# Autodesk Inventor assembly: dog_2
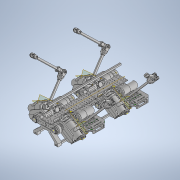
[picture p0: Inventor's stored thumbnail of the model, 180x180]
Saved by Autodesk Inventor 2020 (Build 240168000, 168)
## iProperties
Created: 2019-05-16
Part Number: dog_2
Document SubType Name: Assembly
Designer: psrob
Author: psrob
## Documents named in this file (11)
- E:\projects-2\project dog gen2\hardware\dog_2.iam
- E:\projects-2\project dog gen2\hardware\leg_ass_1.iam
- E:\projects-2\project dog gen2\hardware\carbon_fiber_200.ipt
- E:\projects-2\project dog gen2\hardware\leg_ass_1_MIR.iam
- E:\projects-2\project dog gen2\hardware\body_bone_1.ipt
- E:\projects-2\project dog gen2\hardware\body_bone_2.ipt
- E:\projects-2\project dog gen2\hardware\body_bone_3.ipt
- E:\projects-2\project dog gen2\hardware\body_bone_4.ipt
- E:\projects-2\project dog gen2\hardware\body_bone_5.ipt
- E:\projects-2\project dog gen2\hardware\pcb_shell_ass.iam
- E:\projects-2\project dog gen2\hardware\body_carbon_fiber_holder_1.ipt
## Components (19 placed, 10 different names)
1. leg_ass_1:1 [sub-assembly] — Flush:2, Flush:3, Flush:4, Mate:4, Flush:8, Flush:9, Insert:6, Flush:14, Insert:8, Flush:18
2. leg_ass_1:2 [sub-assembly] — Flush:2, Flush:3, Flush:4, Mate:1, Mate:2, Flush:5, Mate:3, Flush:6, Flush:7, Flush:10, Flush:12, Insert:1, Insert:4, Insert:10, Insert:11, Flush:17, Flush:27
3. carbon_fiber_200:1 — Mate:1, Mate:2, Flush:5, Flush:15, Flush:16
4. leg_ass_1_MIR:1 [sub-assembly] — Mate:3, Flush:6, Flush:7, Insert:2, Insert:3, Flush:13, Insert:9, Insert:12, Flush:20
5. leg_ass_1_MIR:2 [sub-assembly] — Mate:4, Flush:8, Flush:9, Flush:11, Insert:5, Insert:7, Flush:22
6. body_bone_1:1 — Flush:10, Insert:3, Insert:4
7. body_bone_2:1 — Flush:11, Insert:5, Insert:6
8. body_bone_3:1 — Flush:12, Insert:1, Insert:2
9. body_bone_4:1 — Flush:13, Insert:9, Insert:10
10. body_bone_5:1 — Flush:14, Insert:7, Insert:8, Mate:7, Mate:8, Flush:21, Mate:10
11. carbon_fiber_200:2 — Flush:15, Flush:16, Flush:25, Flush:26
12. body_bone_1:2 — Insert:11, Insert:12, Angle:1, Mate:5, Mate:6, Mate:9, Flush:19, Mate:11, Mate:12
13. pcb_shell_ass:1 [sub-assembly] — Flush:17, Angle:1, Mate:5, Mate:6, Flush:24
14. pcb_shell_ass:2 [sub-assembly] — Mate:7, Mate:8, Flush:18
15. pcb_shell_ass:3 [sub-assembly] — Mate:9, Flush:19, Flush:20, Flush:23
16. pcb_shell_ass:4 [sub-assembly] — Flush:21, Mate:10, Flush:22
17. carbon_fiber_200:3 — Flush:23, Mate:11, Flush:25
18. carbon_fiber_200:4 — Flush:24, Mate:12, Flush:26
19. body_carbon_fiber_holder_1:1 — Flush:27
## Relationships (51: Flush 26, Mate 12, Insert 12, Angle 1)
- Flush:2: leg_ass_1:1 ↔ leg_ass_1:2
- Flush:3 (180 mm): leg_ass_1:1 ↔ leg_ass_1:2
- Flush:4: leg_ass_1:1 ↔ leg_ass_1:2
- Mate:1: leg_ass_1:2 ↔ carbon_fiber_200:1
- Mate:2: leg_ass_1:2 ↔ carbon_fiber_200:1
- Flush:5 (10 mm): leg_ass_1:2 ↔ carbon_fiber_200:1
- Mate:3: leg_ass_1:2 ↔ leg_ass_1_MIR:1
- Flush:6: leg_ass_1:2 ↔ leg_ass_1_MIR:1
- Flush:7: leg_ass_1:2 ↔ leg_ass_1_MIR:1
- Mate:4: leg_ass_1:1 ↔ leg_ass_1_MIR:2
- Flush:8: leg_ass_1:1 ↔ leg_ass_1_MIR:2
- Flush:9: leg_ass_1:1 ↔ leg_ass_1_MIR:2
- Flush:10: leg_ass_1:2 ↔ body_bone_1:1
- Flush:11: leg_ass_1_MIR:2 ↔ body_bone_2:1
- Flush:12: leg_ass_1:2 ↔ body_bone_3:1
- Insert:1: leg_ass_1:2 ↔ body_bone_3:1
- Insert:2: leg_ass_1_MIR:1 ↔ body_bone_3:1
- Insert:3: leg_ass_1_MIR:1 ↔ body_bone_1:1
- Insert:4: leg_ass_1:2 ↔ body_bone_1:1
- Insert:5: leg_ass_1_MIR:2 ↔ body_bone_2:1
- Insert:6: leg_ass_1:1 ↔ body_bone_2:1
- Flush:13: leg_ass_1_MIR:1 ↔ body_bone_4:1
- Flush:14: leg_ass_1:1 ↔ body_bone_5:1
- Insert:7: leg_ass_1_MIR:2 ↔ body_bone_5:1
- Insert:8: leg_ass_1:1 ↔ body_bone_5:1
- Insert:9: leg_ass_1_MIR:1 ↔ body_bone_4:1
- Insert:10: leg_ass_1:2 ↔ body_bone_4:1
- Flush:15: carbon_fiber_200:1 ↔ carbon_fiber_200:2
- Flush:16: carbon_fiber_200:1 ↔ carbon_fiber_200:2
- Insert:11: leg_ass_1:2 ↔ body_bone_1:2
- Insert:12: leg_ass_1_MIR:1 ↔ body_bone_1:2
- Flush:17 (10 mm): leg_ass_1:2 ↔ pcb_shell_ass:1
- Angle:1 (180 deg): body_bone_1:2 ↔ pcb_shell_ass:1
- Mate:5 (10 mm): body_bone_1:2 ↔ pcb_shell_ass:1
- Mate:6 (10 mm): body_bone_1:2 ↔ pcb_shell_ass:1
- Mate:7 (10 mm): body_bone_5:1 ↔ pcb_shell_ass:2
- Mate:8 (10 mm): body_bone_5:1 ↔ pcb_shell_ass:2
- Flush:18 (10 mm): leg_ass_1:1 ↔ pcb_shell_ass:2
- Mate:9 (10 mm): body_bone_1:2 ↔ pcb_shell_ass:3
- Flush:19 (10 mm): body_bone_1:2 ↔ pcb_shell_ass:3
- Flush:20 (10 mm): leg_ass_1_MIR:1 ↔ pcb_shell_ass:3
- Flush:21 (10 mm): body_bone_5:1 ↔ pcb_shell_ass:4
- Mate:10 (10 mm): body_bone_5:1 ↔ pcb_shell_ass:4
- Flush:22 (10 mm): leg_ass_1_MIR:2 ↔ pcb_shell_ass:4
- Flush:23 (30 mm): pcb_shell_ass:3 ↔ carbon_fiber_200:3
- Flush:24 (30 mm): pcb_shell_ass:1 ↔ carbon_fiber_200:4
- Mate:11 (40 mm): body_bone_1:2 ↔ carbon_fiber_200:3
- Mate:12 (40 mm): body_bone_1:2 ↔ carbon_fiber_200:4
- Flush:25 (-10 mm): carbon_fiber_200:2 ↔ carbon_fiber_200:3
- Flush:26 (-10 mm): carbon_fiber_200:2 ↔ carbon_fiber_200:4
- Flush:27: leg_ass_1:2 ↔ body_carbon_fiber_holder_1:1
